# Autodesk Inventor assembly: タミヤダンパー1
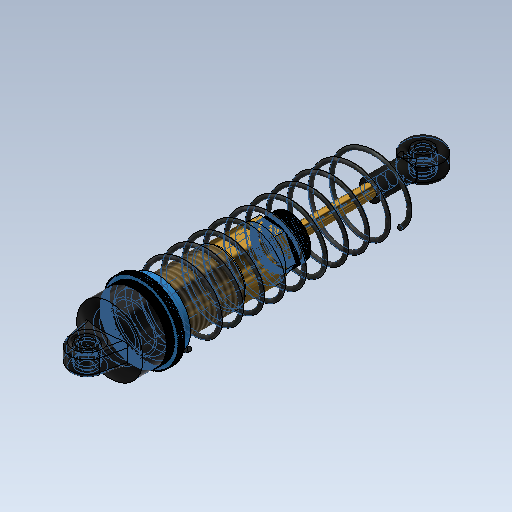
[picture p0: Inventor's stored thumbnail of the model, 512x512]
Saved by Autodesk Inventor 2020 (Build 240168000, 168)
## iProperties
Part Number: タミヤダンパー1
Material: 一般
Document SubType Name: Assembly
Designer: 雪村
Mass: 70.8088 g
Surface Area: 76.0005 cm^2
Volume: 5.6847 cm^3
Density: 12.456 g/cm^3
Author: 雪村
## Documents named in this file (10)
- C:\Users\happy\OneDrive\ドキュメント\賢一ファイル\SRDC\試作10-2\アセンブリ\タミヤダンパー1.iam
- C:\Users\happy\OneDrive\ドキュメント\賢一ファイル\SRDC\試作10-2\ダンパ\タミヤダンパー1.ipt
- C:\Users\happy\OneDrive\ドキュメント\賢一ファイル\SRDC\試作10-2\ダンパ\タミヤダンパー2.ipt
- C:\Users\happy\OneDrive\ドキュメント\賢一ファイル\SRDC\試作10-2\ダンパ\タミヤダンパー3.ipt
- C:\Users\happy\OneDrive\ドキュメント\賢一ファイル\SRDC\試作10-2\ダンパ\タミヤダンパー4.ipt
- C:\Users\happy\OneDrive\ドキュメント\賢一ファイル\SRDC\試作10-2\ダンパ\タミヤダンパー6.ipt
- C:\Users\happy\OneDrive\ドキュメント\賢一ファイル\SRDC\試作10-2\ダンパ\タミヤダンパー5.ipt
- C:\Users\happy\OneDrive\ドキュメント\賢一ファイル\SRDC\試作10-2\ダンパ\タミヤダンパー7.ipt
- C:\Users\happy\OneDrive\ドキュメント\賢一ファイル\SRDC\試作10-2\ダンパ\タミヤダンパー8.ipt
- C:\Users\happy\OneDrive\ドキュメント\賢一ファイル\SRDC\試作10-2\ダンパ\タミヤダンパー9.ipt
## Components (10 placed, 9 different names)
1. タミヤダンパー1:1 — 挿入:1, ボール:2, フラッシュ:1, フラッシュ:3
2. タミヤダンパー2:1 — 挿入:1, 挿入:2, メイト:1, 円柱状:2
3. タミヤダンパー3:1 — 挿入:2, 挿入:3
4. タミヤダンパー4:1 — メイト:1, 円柱状:2
5. タミヤダンパー6:1 — 挿入:3, メイト:2
6. タミヤダンパー5:1 — 挿入:4, メイト:2, メイト:3
7. タミヤダンパー7:1 — 挿入:4, ボール:1, フラッシュ:1
8. タミヤダンパー8:1 — ボール:2, フラッシュ:2, フラッシュ:3
9. タミヤダンパー8:2 — ボール:1, フラッシュ:2
10. タミヤダンパー9:1 — メイト:3
## Relationships (13: Insert 4, Mate 3, Flush 3, BallJoint 2, CylindricalJoint 1)
- 挿入:1 [Insert]: タミヤダンパー1:1 ↔ タミヤダンパー2:1
- 挿入:2 [Insert]: タミヤダンパー2:1 ↔ タミヤダンパー3:1
- メイト:1 [Mate]: タミヤダンパー2:1 ↔ タミヤダンパー4:1
- 挿入:3 [Insert]: タミヤダンパー3:1 ↔ タミヤダンパー6:1
- 挿入:4 [Insert] (-3 mm): タミヤダンパー5:1 ↔ タミヤダンパー7:1
- ボール:1 [BallJoint]: タミヤダンパー7:1 ↔ タミヤダンパー8:2
- ボール:2 [BallJoint]: タミヤダンパー1:1 ↔ タミヤダンパー8:1
- フラッシュ:1 [Flush]: タミヤダンパー1:1 ↔ タミヤダンパー7:1
- 円柱状:2 [CylindricalJoint]: タミヤダンパー2:1 ↔ タミヤダンパー4:1
- フラッシュ:2 [Flush]: タミヤダンパー8:1 ↔ タミヤダンパー8:2
- フラッシュ:3 [Flush]: タミヤダンパー1:1 ↔ タミヤダンパー8:1
- メイト:2 [Mate]: タミヤダンパー6:1 ↔ タミヤダンパー5:1
- メイト:3 [Mate]: タミヤダンパー5:1 ↔ タミヤダンパー9:1
